# Autodesk Inventor assembly: rollertriangleassembly
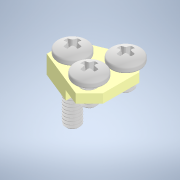
[picture p0: Inventor's stored thumbnail of the model, 180x180]
Saved by Autodesk Inventor 2022 (Build 260153000, 153)
## iProperties
Created: 2022-11-07
Part Number: rollertriangleassembly
Document SubType Name: Assembly
Designer: matia
Author: matia
## Documents named in this file (4)
- C:\Users\matia\Desktop\1QuadMod\rollertriangleassembly.iam
- C:\Users\matia\Desktop\1QuadMod\rollertriangle(v3).ipt
- C:\Users\matia\Desktop\1QuadMod\91772A123_Passivated 18-8 Stainless Steel Pan Head Phillips Screw.ipt
- C:\Users\matia\Desktop\1QuadMod\91772A128_Passivated 18-8 Stainless Steel Pan Head Phillips Screw.ipt
## Components (4 placed, 3 different names)
1. rollertriangle(v3):1 — Mate:1, Mate:2, Mate:3, Mate:4, Rotation:1
2. 91772A123_Passivated 18-8 Stainless Steel Pan Head Phillips Screw:1 — Mate:1
3. 91772A123_Passivated 18-8 Stainless Steel Pan Head Phillips Screw:2 — Mate:2, Rotation:1
4. 91772A128_Passivated 18-8 Stainless Steel Pan Head Phillips Screw:1 — Mate:3, Mate:4
## Relationships (5: Mate 4, RelateRotation 1)
- Mate:1: rollertriangle(v3):1 ↔ 91772A123_Passivated 18-8 Stainless Steel Pan Head Phillips Screw:1
- Mate:2: rollertriangle(v3):1 ↔ 91772A123_Passivated 18-8 Stainless Steel Pan Head Phillips Screw:2
- Mate:3: rollertriangle(v3):1 ↔ 91772A128_Passivated 18-8 Stainless Steel Pan Head Phillips Screw:1
- Mate:4: rollertriangle(v3):1 ↔ 91772A128_Passivated 18-8 Stainless Steel Pan Head Phillips Screw:1
- Rotation:1 [RelateRotation] (1 ul): rollertriangle(v3):1 ↔ 91772A123_Passivated 18-8 Stainless Steel Pan Head Phillips Screw:2
